# Autodesk Inventor assembly: Trunk
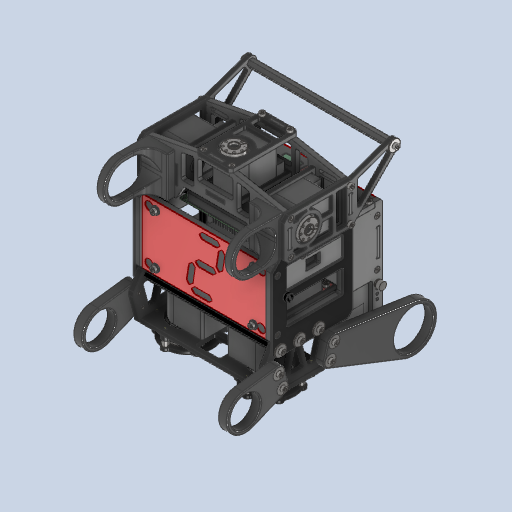
[picture p0: Inventor's stored thumbnail of the model, 512x512]
Saved by Autodesk Inventor 2022.5 (Build 265521000, 521)
## iProperties
Created: 2022-01-06
Part Number: Trunk
Document SubType Name: Assembly
Designer: Masato Kubotera
Mass: 836.462 g
Surface Area: 2738.45 cm^2
Volume: 519.507 cm^3
Density: 1.61011 g/cm^3
Author: Masato Kubotera
## Documents named in this file (26)
- C:\Users\Masato\Documents\Inventor\SUSTAINA-OP\ModelingFiles\UpperBody\Trunk\Trunk.iam
- C:\Users\Masato\Documents\Inventor\SUSTAINA-OP\ModelingFiles\COTS\KONDO\B3M-SC-1170-A.ipt
- C:\Users\Masato\Documents\Inventor\SUSTAINA-OP\ModelingFiles\UpperBody\Trunk\Trunk_neck_frame.ipt
- C:\Users\Masato\Documents\Inventor\SUSTAINA-OP\ModelingFiles\COTS\Screw\FC-2615EB.ipt
- C:\Users\Masato\Documents\Inventor\SUSTAINA-OP\ModelingFiles\COTS\Screw\UC-0306.ipt
- C:\Users\Masato\Documents\Inventor\SUSTAINA-OP\ModelingFiles\COTS\Screw\UC-0308.ipt
- C:\Users\Masato\Documents\Inventor\SUSTAINA-OP\ModelingFiles\UpperBody\Trunk\Trunk_shoulder_frame.ipt
- C:\Users\Masato\Documents\Inventor\SUSTAINA-OP\ModelingFiles\UpperBody\Trunk\Trunk_upper_side_frame.ipt
- C:\Users\Masato\Documents\Inventor\SUSTAINA-OP\ModelingFiles\COTS\Screw\UC-0310.ipt
- C:\Users\Masato\Documents\Inventor\SUSTAINA-OP\ModelingFiles\UpperBody\Trunk\Trunk_shoulder_frame_MIR.ipt
- C:\Users\Masato\Documents\Inventor\SUSTAINA-OP\ModelingFiles\COTS\Washer\UUW-0312-10H.ipt
- C:\Users\Masato\Documents\Inventor\SUSTAINA-OP\ModelingFiles\UpperBody\Trunk\Trunk_lower_side_frame.ipt
- C:\Users\Masato\Documents\Inventor\SUSTAINA-OP\ModelingFiles\UpperBody\Trunk\Trunk_waisit_frame.ipt
- C:\Users\Masato\Documents\Inventor\SUSTAINA-OP\ModelingFiles\UpperBody\Trunk\CrossRollerBearing\BearingUnit.iam
- C:\Users\Masato\Documents\Inventor\SUSTAINA-OP\ModelingFiles\COTS\Screw\CSMKN-SUSTBS-M3-6.ipt
- C:\Users\Masato\Documents\Inventor\SUSTAINA-OP\ModelingFiles\COTS\Spacer\ABLSBF7-140-M3-N3.ipt
- C:\Users\Masato\Documents\Inventor\SUSTAINA-OP\ModelingFiles\COTS\Spacer\SLSBF7-157-M3-N3.ipt
- C:\Users\Masato\Documents\Inventor\SUSTAINA-OP\ModelingFiles\COTS\Spacer\BRU-309S.ipt
- C:\Users\Masato\Documents\Inventor\SUSTAINA-OP\ModelingFiles\UpperBody\Trunk\Trunk_servo_bottom_frame.ipt
- C:\Users\Masato\Documents\Inventor\SUSTAINA-OP\ModelingFiles\COTS\KONDO\B3M-SC-1040-A_with_ClampHorn.iam
- C:\Users\Masato\Documents\Inventor\SUSTAINA-OP\ModelingFiles\UpperBody\Trunk\FrontBumper.ipt
- C:\Users\Masato\Documents\Inventor\SUSTAINA-OP\ModelingFiles\UpperBody\Trunk\RearBumper.ipt
- C:\Users\Masato\Documents\Inventor\SUSTAINA-OP\ModelingFiles\UpperBody\Trunk\ChestBumper.ipt
- C:\Users\Masato\Documents\Inventor\SUSTAINA-OP\ModelingFiles\UpperBody\Trunk\Handle_ShrinkTube.ipt
- C:\Users\Masato\Documents\Inventor\SUSTAINA-OP\ModelingFiles\UpperBody\Trunk\Trunk_chest_frame.iam
- C:\Users\Masato\Documents\Inventor\SUSTAINA-OP\ModelingFiles\UpperBody\Cockpit\Cockpit.iam
## Components (93 placed, 25 different names)
1. BearingUnit:1 [sub-assembly] — 挿入:23, 挿入:24
2. BearingUnit:2 [sub-assembly] — 挿入:25, 挿入:26
3. Trunk_chest_frame:1 [sub-assembly] — Insert:107, Insert:108, Insert:112, Insert:113, Insert:114, Insert:115, メイト:15, メイト:16, フラッシュ:15, フラッシュ:16
4. Trunk_chest_frame:2 [sub-assembly] — Insert:109, Insert:110, Insert:116, Insert:117, Insert:118, Insert:119
5. Cockpit:1 [sub-assembly] — 挿入:251, 角度:12
6. Trunk_shoulder_frame:1 — 挿入:5, 挿入:6, 挿入:7, 挿入:8, 挿入:9, 挿入:10, 挿入:11, 挿入:12, 挿入:50, メイト:3, Insert:120
7. Trunk_shoulder_frame_MIR:1 — 挿入:13, 挿入:14, 挿入:15, 挿入:16, 挿入:17, 挿入:18, 挿入:19, 挿入:20, 角度:1, 挿入:52, Insert:121
8. Trunk_upper_side_frame:1 — 挿入:5, 挿入:6, 挿入:7, 挿入:8, 挿入:35, 挿入:82, 挿入:83, メイト:2, 挿入:100, 挿入:101, 挿入:102, Insert:112, Insert:113, Insert:116, Insert:117, メイト:17, 挿入:251
9. Trunk_upper_side_frame:2 — 挿入:13, 挿入:14, 挿入:15, 挿入:16, 挿入:36, メイト:1, 挿入:103, 挿入:104, 挿入:105, Insert:114, Insert:115, Insert:118, Insert:119, メイト:18
10. Trunk_neck_frame:1 — 挿入:1, 挿入:2, 挿入:3, 挿入:4, Insert:107, Insert:108, Insert:109, Insert:110, Insert:111, Flush:7
11. Trunk_waisit_frame:1 — フラッシュ:1, フラッシュ:2, フラッシュ:3, 挿入:23, 挿入:24, 挿入:25, 挿入:26, 挿入:27, 挿入:28, 挿入:29, 挿入:30, 挿入:31, 挿入:32, 挿入:33, 挿入:34, 挿入:37, 挿入:38, 挿入:39, 挿入:40, 挿入:54, 挿入:55, 挿入:72, 挿入:73
12. Trunk_lower_side_frame:1 — 挿入:72, 挿入:73, 角度:2, 角度:3, 挿入:74, 挿入:75, 挿入:82, 挿入:83, 挿入:88, 挿入:89, 挿入:90, 挿入:91
13. Trunk_lower_side_frame:2 — 挿入:54, 挿入:55, 挿入:84, 挿入:85, 挿入:86, 挿入:87
14. Trunk_servo_bottom_frame:1 — 挿入:106, Flush:6
15. Trunk_servo_bottom_frame:2 — Insert:122, Angle:6
16. Trunk_servo_bottom_frame:3 — Insert:123, Angle:7
17. ChestBumper:1 — メイト:1, メイト:16, メイト:18, フラッシュ:16
18. ChestBumper:2 — メイト:2, メイト:15, メイト:17, フラッシュ:15
19. RearBumper:1 — 挿入:94, 挿入:95
20. RearBumper:2 — 挿入:98, 挿入:99
21. FrontBumper:1 — 挿入:92, 挿入:93
22. FrontBumper:2 — 挿入:96, 挿入:97
23. BRU-309S:1 — 挿入:56, 挿入:88
24. BRU-309S:2 — 挿入:57, 挿入:89
25. BRU-309S:3 — 挿入:58, 挿入:90
26. BRU-309S:4 — 挿入:59, 挿入:91
27. BRU-309S:5 — 挿入:60, 挿入:84
28. BRU-309S:6 — 挿入:61, 挿入:85
29. BRU-309S:7 — 挿入:62, 挿入:86
30. BRU-309S:8 — 挿入:63, 挿入:87
31. UUW-0312-10H:1 — 挿入:21, 挿入:51
32. UUW-0312-10H:2 — 挿入:22, 挿入:53
33. UUW-0312-10H:11 — 挿入:56, 挿入:64, 挿入:92
34. UUW-0312-10H:12 — 挿入:57, 挿入:65, 挿入:93
35. UUW-0312-10H:13 — 挿入:58, 挿入:66, 挿入:94
36. UUW-0312-10H:14 — 挿入:59, 挿入:67, 挿入:95
37. UUW-0312-10H:15 — 挿入:60, 挿入:68, 挿入:98
38. UUW-0312-10H:16 — 挿入:61, 挿入:69, 挿入:99
39. UUW-0312-10H:17 — 挿入:62, 挿入:70, 挿入:96
40. UUW-0312-10H:18 — 挿入:63, 挿入:71, 挿入:97
41. UUW-0312-10H:19 — 挿入:76, 挿入:100
42. UUW-0312-10H:20 — 挿入:80, 挿入:101
43. UUW-0312-10H:21 — 挿入:77, 挿入:102
44. UUW-0312-10H:22 — 挿入:78, 挿入:103
45. UUW-0312-10H:23 — 挿入:81, 挿入:104
46. UUW-0312-10H:24 — 挿入:79, 挿入:105
47. SLSBF7-157-M3-N3:1 — 角度:1, 挿入:50, 挿入:51, 挿入:52, 挿入:53, フラッシュ:4, フラッシュ:5
48. ABLSBF7-140-M3-N3:1 — 角度:2, 挿入:74
49. ABLSBF7-140-M3-N3:2 — 角度:3, 挿入:75
50. B3M-SC-1170-A:1 — 挿入:27, 挿入:28
51. B3M-SC-1170-A:2 — 挿入:29, 挿入:30
52. B3M-SC-1040-A_with_ClampHorn:1 [sub-assembly] — 挿入:106, Mate:3, Insert:111
53. B3M-SC-1040-A_with_ClampHorn:2 [sub-assembly] — Insert:120, Angle:4, Insert:122
54. B3M-SC-1040-A_with_ClampHorn:3 [sub-assembly] — Insert:121, Angle:5, Insert:123
55. Handle_ShrinkTube:1 — フラッシュ:4, フラッシュ:5, メイト:3
56. UC-0306:9 — 挿入:64
57. UC-0306:10 — 挿入:65
58. UC-0306:11 — 挿入:66
59. UC-0306:12 — 挿入:67
60. UC-0306:13 — 挿入:68
61. UC-0306:14 — 挿入:69
62. UC-0306:15 — 挿入:71
63. UC-0306:16 — 挿入:70
64. UC-0310:17 — 挿入:76
65. UC-0310:18 — 挿入:77
66. UC-0310:19 — 挿入:78
67. UC-0310:20 — 挿入:79
68. UC-0308:7 — 挿入:80
69. UC-0308:8 — 挿入:81
70. UC-0310:13 — 挿入:37
71. UC-0310:14 — 挿入:38
72. UC-0310:15 — 挿入:39
73. UC-0310:16 — 挿入:40
74. CSMKN-SUSTBS-M3-6:1 — 挿入:35
75. CSMKN-SUSTBS-M3-6:2 — 挿入:36
76. UC-0308:2 — 挿入:4
77. UC-0308:1 — 挿入:3
78. UC-0306:2 — 挿入:2
79. UC-0306:1 — 挿入:1
80. UC-0308:4 — 挿入:11
81. UC-0308:3 — 挿入:9
82. UC-0310:4 — 挿入:12
83. UC-0310:3 — 挿入:10
84. UC-0310:6 — 挿入:20
85. UC-0310:5 — 挿入:19
86. UC-0308:6 — 挿入:18
87. UC-0308:5 — 挿入:17
88. UC-0306:4 — 挿入:22
89. UC-0306:3 — 挿入:21
90. FC-2615EB:16 — 挿入:34
91. FC-2615EB:15 — 挿入:33
92. FC-2615EB:14 — 挿入:32
93. FC-2615EB:13 — 挿入:31
## Relationships (140: Insert 115, Flush 9, Angle 8, Mate 8)
- 挿入:1 [Insert]: Trunk_neck_frame:1 ↔ UC-0306:1
- 挿入:2 [Insert]: Trunk_neck_frame:1 ↔ UC-0306:2
- 挿入:3 [Insert]: Trunk_neck_frame:1 ↔ UC-0308:1
- 挿入:4 [Insert]: Trunk_neck_frame:1 ↔ UC-0308:2
- 挿入:5 [Insert]: Trunk_shoulder_frame:1 ↔ Trunk_upper_side_frame:1
- 挿入:6 [Insert]: Trunk_shoulder_frame:1 ↔ Trunk_upper_side_frame:1
- 挿入:7 [Insert]: Trunk_shoulder_frame:1 ↔ Trunk_upper_side_frame:1
- 挿入:8 [Insert]: Trunk_shoulder_frame:1 ↔ Trunk_upper_side_frame:1
- 挿入:9 [Insert]: Trunk_shoulder_frame:1 ↔ UC-0308:3
- 挿入:10 [Insert]: Trunk_shoulder_frame:1 ↔ UC-0310:3
- 挿入:11 [Insert]: Trunk_shoulder_frame:1 ↔ UC-0308:4
- 挿入:12 [Insert]: Trunk_shoulder_frame:1 ↔ UC-0310:4
- 挿入:13 [Insert]: Trunk_shoulder_frame_MIR:1 ↔ Trunk_upper_side_frame:2
- 挿入:14 [Insert]: Trunk_shoulder_frame_MIR:1 ↔ Trunk_upper_side_frame:2
- 挿入:15 [Insert]: Trunk_shoulder_frame_MIR:1 ↔ Trunk_upper_side_frame:2
- 挿入:16 [Insert]: Trunk_shoulder_frame_MIR:1 ↔ Trunk_upper_side_frame:2
- 挿入:17 [Insert]: Trunk_shoulder_frame_MIR:1 ↔ UC-0308:5
- 挿入:18 [Insert]: Trunk_shoulder_frame_MIR:1 ↔ UC-0308:6
- 挿入:19 [Insert]: Trunk_shoulder_frame_MIR:1 ↔ UC-0310:5
- 挿入:20 [Insert]: Trunk_shoulder_frame_MIR:1 ↔ UC-0310:6
- 挿入:21 [Insert]: UUW-0312-10H:1 ↔ UC-0306:3
- 挿入:22 [Insert]: UUW-0312-10H:2 ↔ UC-0306:4
- フラッシュ:1 [Flush]: Trunk_waisit_frame:1
- フラッシュ:2 [Flush]: Trunk_waisit_frame:1
- フラッシュ:3 [Flush]: Trunk_waisit_frame:1
- 挿入:23 [Insert]: BearingUnit:1 ↔ Trunk_waisit_frame:1
- 挿入:24 [Insert]: BearingUnit:1 ↔ Trunk_waisit_frame:1
- 挿入:25 [Insert]: BearingUnit:2 ↔ Trunk_waisit_frame:1
- 挿入:26 [Insert]: BearingUnit:2 ↔ Trunk_waisit_frame:1
- 挿入:27 [Insert]: Trunk_waisit_frame:1 ↔ B3M-SC-1170-A:1
- 挿入:28 [Insert]: Trunk_waisit_frame:1 ↔ B3M-SC-1170-A:1
- 挿入:29 [Insert]: Trunk_waisit_frame:1 ↔ B3M-SC-1170-A:2
- 挿入:30 [Insert]: Trunk_waisit_frame:1 ↔ B3M-SC-1170-A:2
- 挿入:31 [Insert]: Trunk_waisit_frame:1 ↔ FC-2615EB:13
- 挿入:32 [Insert]: Trunk_waisit_frame:1 ↔ FC-2615EB:14
- 挿入:33 [Insert]: Trunk_waisit_frame:1 ↔ FC-2615EB:15
- 挿入:34 [Insert]: Trunk_waisit_frame:1 ↔ FC-2615EB:16
- 挿入:35 [Insert]: Trunk_upper_side_frame:1 ↔ CSMKN-SUSTBS-M3-6:1
- 挿入:36 [Insert]: Trunk_upper_side_frame:2 ↔ CSMKN-SUSTBS-M3-6:2
- 挿入:37 [Insert]: Trunk_waisit_frame:1 ↔ UC-0310:13
- 挿入:38 [Insert]: Trunk_waisit_frame:1 ↔ UC-0310:14
- 挿入:39 [Insert]: Trunk_waisit_frame:1 ↔ UC-0310:15
- 挿入:40 [Insert]: Trunk_waisit_frame:1 ↔ UC-0310:16
- 角度:1 [Angle] (0 deg): Trunk_shoulder_frame_MIR:1 ↔ SLSBF7-157-M3-N3:1
- 挿入:50 [Insert]: Trunk_shoulder_frame:1 ↔ SLSBF7-157-M3-N3:1
- 挿入:51 [Insert]: UUW-0312-10H:1 ↔ SLSBF7-157-M3-N3:1
- 挿入:52 [Insert]: Trunk_shoulder_frame_MIR:1 ↔ SLSBF7-157-M3-N3:1
- 挿入:53 [Insert]: UUW-0312-10H:2 ↔ SLSBF7-157-M3-N3:1
- 挿入:54 [Insert]: Trunk_waisit_frame:1 ↔ Trunk_lower_side_frame:2
- 挿入:55 [Insert]: Trunk_waisit_frame:1 ↔ Trunk_lower_side_frame:2
- 挿入:56 [Insert]: BRU-309S:1 ↔ UUW-0312-10H:11
- 挿入:57 [Insert]: BRU-309S:2 ↔ UUW-0312-10H:12
- 挿入:58 [Insert]: BRU-309S:3 ↔ UUW-0312-10H:13
- 挿入:59 [Insert]: BRU-309S:4 ↔ UUW-0312-10H:14
- 挿入:60 [Insert]: BRU-309S:5 ↔ UUW-0312-10H:15
- 挿入:61 [Insert]: BRU-309S:6 ↔ UUW-0312-10H:16
- 挿入:62 [Insert]: BRU-309S:7 ↔ UUW-0312-10H:17
- 挿入:63 [Insert]: BRU-309S:8 ↔ UUW-0312-10H:18
- 挿入:64 [Insert]: UUW-0312-10H:11 ↔ UC-0306:9
- 挿入:65 [Insert]: UUW-0312-10H:12 ↔ UC-0306:10
- 挿入:66 [Insert]: UUW-0312-10H:13 ↔ UC-0306:11
- 挿入:67 [Insert]: UUW-0312-10H:14 ↔ UC-0306:12
- 挿入:68 [Insert]: UUW-0312-10H:15 ↔ UC-0306:13
- 挿入:69 [Insert]: UUW-0312-10H:16 ↔ UC-0306:14
- 挿入:70 [Insert]: UUW-0312-10H:17 ↔ UC-0306:16
- 挿入:71 [Insert]: UUW-0312-10H:18 ↔ UC-0306:15
- 挿入:72 [Insert]: Trunk_waisit_frame:1 ↔ Trunk_lower_side_frame:1
- 挿入:73 [Insert]: Trunk_waisit_frame:1 ↔ Trunk_lower_side_frame:1
- 角度:2 [Angle] (0 deg): Trunk_lower_side_frame:1 ↔ ABLSBF7-140-M3-N3:1
- 角度:3 [Angle] (0 deg): Trunk_lower_side_frame:1 ↔ ABLSBF7-140-M3-N3:2
- 挿入:74 [Insert]: Trunk_lower_side_frame:1 ↔ ABLSBF7-140-M3-N3:1
- 挿入:75 [Insert]: Trunk_lower_side_frame:1 ↔ ABLSBF7-140-M3-N3:2
- 挿入:76 [Insert]: UUW-0312-10H:19 ↔ UC-0310:17
- 挿入:77 [Insert]: UUW-0312-10H:21 ↔ UC-0310:18
- 挿入:78 [Insert]: UUW-0312-10H:22 ↔ UC-0310:19
- 挿入:79 [Insert]: UUW-0312-10H:24 ↔ UC-0310:20
- 挿入:80 [Insert]: UUW-0312-10H:20 ↔ UC-0308:7
- 挿入:81 [Insert]: UUW-0312-10H:23 ↔ UC-0308:8
- 挿入:82 [Insert]: Trunk_upper_side_frame:1 ↔ Trunk_lower_side_frame:1
- 挿入:83 [Insert]: Trunk_upper_side_frame:1 ↔ Trunk_lower_side_frame:1
- 挿入:84 [Insert]: Trunk_lower_side_frame:2 ↔ BRU-309S:5
- 挿入:85 [Insert]: Trunk_lower_side_frame:2 ↔ BRU-309S:6
- 挿入:86 [Insert]: Trunk_lower_side_frame:2 ↔ BRU-309S:7
- 挿入:87 [Insert]: Trunk_lower_side_frame:2 ↔ BRU-309S:8
- 挿入:88 [Insert]: Trunk_lower_side_frame:1 ↔ BRU-309S:1
- 挿入:89 [Insert]: Trunk_lower_side_frame:1 ↔ BRU-309S:2
- 挿入:90 [Insert]: Trunk_lower_side_frame:1 ↔ BRU-309S:3
- 挿入:91 [Insert]: Trunk_lower_side_frame:1 ↔ BRU-309S:4
- 挿入:92 [Insert]: FrontBumper:1 ↔ UUW-0312-10H:11
- 挿入:93 [Insert]: FrontBumper:1 ↔ UUW-0312-10H:12
- 挿入:94 [Insert]: RearBumper:1 ↔ UUW-0312-10H:13
- 挿入:95 [Insert]: RearBumper:1 ↔ UUW-0312-10H:14
- 挿入:96 [Insert]: FrontBumper:2 ↔ UUW-0312-10H:17
- 挿入:97 [Insert]: FrontBumper:2 ↔ UUW-0312-10H:18
- 挿入:98 [Insert]: RearBumper:2 ↔ UUW-0312-10H:15
- 挿入:99 [Insert]: RearBumper:2 ↔ UUW-0312-10H:16
- メイト:1 [Mate]: Trunk_upper_side_frame:2 ↔ ChestBumper:1
- メイト:2 [Mate]: Trunk_upper_side_frame:1 ↔ ChestBumper:2
- 挿入:100 [Insert]: Trunk_upper_side_frame:1 ↔ UUW-0312-10H:19
- 挿入:101 [Insert]: Trunk_upper_side_frame:1 ↔ UUW-0312-10H:20
- 挿入:102 [Insert]: Trunk_upper_side_frame:1 ↔ UUW-0312-10H:21
- 挿入:103 [Insert]: Trunk_upper_side_frame:2 ↔ UUW-0312-10H:22
- 挿入:104 [Insert]: Trunk_upper_side_frame:2 ↔ UUW-0312-10H:23
- 挿入:105 [Insert]: Trunk_upper_side_frame:2 ↔ UUW-0312-10H:24
- フラッシュ:4 [Flush]: SLSBF7-157-M3-N3:1 ↔ Handle_ShrinkTube:1
- フラッシュ:5 [Flush]: SLSBF7-157-M3-N3:1 ↔ Handle_ShrinkTube:1
- メイト:3 [Mate]: Trunk_shoulder_frame:1 ↔ Handle_ShrinkTube:1
- 挿入:106 [Insert]: Trunk_servo_bottom_frame:1 ↔ B3M-SC-1040-A_with_ClampHorn:1
- Mate:3: B3M-SC-1040-A_with_ClampHorn:1
- Insert:107: Trunk_chest_frame:1 ↔ Trunk_neck_frame:1
- Insert:108: Trunk_chest_frame:1 ↔ Trunk_neck_frame:1
- Insert:109: Trunk_chest_frame:2 ↔ Trunk_neck_frame:1
- Insert:110: Trunk_chest_frame:2 ↔ Trunk_neck_frame:1
- Insert:111: Trunk_neck_frame:1 ↔ B3M-SC-1040-A_with_ClampHorn:1
- Flush:6: Trunk_servo_bottom_frame:1
- Flush:7: Trunk_neck_frame:1
- Insert:112: Trunk_chest_frame:1 ↔ Trunk_upper_side_frame:1
- Insert:113: Trunk_chest_frame:1 ↔ Trunk_upper_side_frame:1
- Insert:114: Trunk_chest_frame:1 ↔ Trunk_upper_side_frame:2
- Insert:115: Trunk_chest_frame:1 ↔ Trunk_upper_side_frame:2
- Insert:116: Trunk_chest_frame:2 ↔ Trunk_upper_side_frame:1
- Insert:117: Trunk_chest_frame:2 ↔ Trunk_upper_side_frame:1
- Insert:118: Trunk_chest_frame:2 ↔ Trunk_upper_side_frame:2
- Insert:119: Trunk_chest_frame:2 ↔ Trunk_upper_side_frame:2
- Insert:120: Trunk_shoulder_frame:1 ↔ B3M-SC-1040-A_with_ClampHorn:2
- Insert:121: Trunk_shoulder_frame_MIR:1 ↔ B3M-SC-1040-A_with_ClampHorn:3
- Angle:4 (0 deg): B3M-SC-1040-A_with_ClampHorn:2
- Angle:5 (0 deg): B3M-SC-1040-A_with_ClampHorn:3
- Insert:122: Trunk_servo_bottom_frame:2 ↔ B3M-SC-1040-A_with_ClampHorn:2
- Insert:123: Trunk_servo_bottom_frame:3 ↔ B3M-SC-1040-A_with_ClampHorn:3
- Angle:6 (0 deg): Trunk_servo_bottom_frame:2
- Angle:7 (0 deg): Trunk_servo_bottom_frame:3
- メイト:15 [Mate]: Trunk_chest_frame:1 ↔ ChestBumper:2
- メイト:16 [Mate]: Trunk_chest_frame:1 ↔ ChestBumper:1
- メイト:17 [Mate]: Trunk_upper_side_frame:1 ↔ ChestBumper:2
- メイト:18 [Mate]: Trunk_upper_side_frame:2 ↔ ChestBumper:1
- フラッシュ:15 [Flush]: Trunk_chest_frame:1 ↔ ChestBumper:2
- フラッシュ:16 [Flush]: Trunk_chest_frame:1 ↔ ChestBumper:1
- 挿入:251 [Insert]: Cockpit:1 ↔ Trunk_upper_side_frame:1
- 角度:12 [Angle] (0 deg): Cockpit:1
